# Autodesk Inventor assembly: MGN12H Block_MIR
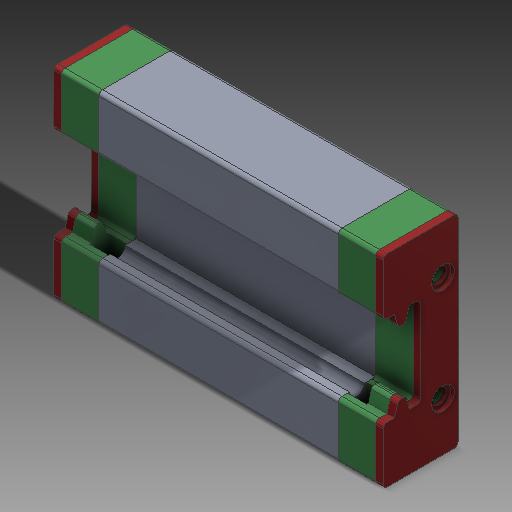
[picture p0: Inventor's stored thumbnail of the model, 512x512]
Saved by Autodesk Inventor 2017.3 (Build 213256000, 256)
## iProperties
Created: 2018-10-07
Part Number: MGN12H Block_MIR
Document SubType Name: Assembly
Designer: Ax
Author: Ax
## Documents named in this file (4)
- C:\Users\Ax\Documents\Inventor\Drakon\Library\mgn12-sliding-block-linear-guide-1.snapshot.2\MGN12H Block_MIR.iam
- C:\Users\Ax\Documents\Inventor\Drakon\Library\mgn12-sliding-block-linear-guide-1.snapshot.2\Main Block_MIR.ipt
- C:\Users\Ax\Documents\Inventor\Drakon\Library\mgn12-sliding-block-linear-guide-1.snapshot.2\Green End Cap_MIR.ipt
- C:\Users\Ax\Documents\Inventor\Drakon\Library\mgn12-sliding-block-linear-guide-1.snapshot.2\Red End Cap_MIR.ipt
## Components (5 placed, 3 different names)
1. Main Block_MIR:1 — Mate:8, Mate:6, Mate:5, Mate:7, Mate:3, Mate:2
2. Green End Cap_MIR:1 — Mate:8, Mate:6, Mate:5, Mate:11, Mate:10, Mate:9
3. Red End Cap_MIR:1 — Mate:11, Mate:10, Mate:9
4. Green End Cap_MIR:2 — Mate:7, Mate:3, Mate:2, Mate:14, Mate:13, Mate:12
5. Red End Cap_MIR:2 — Mate:14, Mate:13, Mate:12
## Relationships (12: Mate 12)
- Mate:8: Main Block_MIR:1 ↔ Green End Cap_MIR:1
- Mate:6: Main Block_MIR:1 ↔ Green End Cap_MIR:1
- Mate:5: Main Block_MIR:1 ↔ Green End Cap_MIR:1
- Mate:11: Green End Cap_MIR:1 ↔ Red End Cap_MIR:1
- Mate:10: Green End Cap_MIR:1 ↔ Red End Cap_MIR:1
- Mate:9: Green End Cap_MIR:1 ↔ Red End Cap_MIR:1
- Mate:7: Main Block_MIR:1 ↔ Green End Cap_MIR:2
- Mate:3: Main Block_MIR:1 ↔ Green End Cap_MIR:2
- Mate:2: Main Block_MIR:1 ↔ Green End Cap_MIR:2
- Mate:14: Green End Cap_MIR:2 ↔ Red End Cap_MIR:2
- Mate:13: Green End Cap_MIR:2 ↔ Red End Cap_MIR:2
- Mate:12: Green End Cap_MIR:2 ↔ Red End Cap_MIR:2
